# Autodesk Inventor assembly: ChassisComplete_NERDS
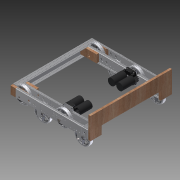
[picture p0: Inventor's stored thumbnail of the model, 180x180]
Saved by Autodesk Inventor 2014 (Build 180170000, 170)
## iProperties
Created: 2016-01-19
Part Number: ChassisComplete_NERDS
Document SubType Name: Assembly
Designer: choices
Author: choices
## Documents named in this file (15)
- C:\Users\choices.CTE\Documents\Nerds_1726\Models\2015-2016\Assemblies\Robot\Chassis.iam
- C:\Users\choices.CTE\Documents\Nerds_1726\Models\2015-2016\AndyMark\6 HiGrip with hub and double pulley.iam
- C:\Users\choices.CTE\Documents\Nerds_1726\Models\2015-2016\AndyMark\FR8ZZ Hex Bearing.ipt
- C:\Users\choices.CTE\Documents\Nerds_1726\Models\2015-2016\AndyMark\am-2598_107 2016 KOP Toughbox Mini.iam
- C:\Users\choices.CTE\Documents\Nerds_1726\Models\2015-2016\AndyMark\6 HiGrip with bearings, pulleys and spacers.iam
- C:\Users\choices.CTE\Documents\Nerds_1726\Models\2015-2016\Parts\Robot\Chassis\FrameInnerRight.ipt
- C:\Users\choices.CTE\Documents\Nerds_1726\Models\2015-2016\AndyMark\375-16 x 4.25 Hex Bolt_HFBOLT 0.375-16x2.5x1-C.ipt
- C:\Users\choices.CTE\Documents\Nerds_1726\Models\2015-2016\Parts\Robot\Chassis\FrameOuterRight.ipt
- C:\Users\choices.CTE\Documents\Nerds_1726\Models\2015-2016\Parts\Robot\Chassis\FrameOuterLeft.ipt
- C:\Users\choices.CTE\Documents\Nerds_1726\Models\2015-2016\Parts\Robot\Chassis\FrameInnerLeft.ipt
- C:\Users\choices.CTE\Documents\Nerds_1726\Models\2015-2016\Parts\Robot\Chassis\DriveFrameEndCaps.ipt
- C:\Users\choices.CTE\Documents\Nerds_1726\Models\2015-2016\Parts\Robot\Chassis\DriveMotor.ipt
- C:\Users\choices.CTE\Documents\Nerds_1726\Models\2015-2016\Parts\Robot\Chassis\BumperMount.ipt
- C:\Users\choices.CTE\Documents\Nerds_1726\Models\2015-2016\Parts\Robot\Chassis\FrameEndSpacer.ipt
- C:\Users\choices.CTE\Documents\Nerds_1726\Models\2015-2016\AndyMark\Chass_EndSheet.ipt
## Components (30 placed, 14 different names)
1. 6 HiGrip with hub and double pulley:1 [sub-assembly] — Mate:7, Mate:8, Mate:9
2. am-2598_107 2016 KOP Toughbox Mini:1 [sub-assembly] — Mate:8, Mate:9, Mate:12, Mate:14, Flush:1, Mate:15, Mate:16, Mate:17, Insert:19, Insert:20
3. FR8ZZ Hex Bearing:1 — Mate:7, Mate:12, Mate:14, Flush:1, Mate:18, Mate:19
4. 6 HiGrip with bearings, pulleys and spacers:1 [sub-assembly] — Insert:5, Tangent:1
5. FrameInnerRight:1 — Mate:15, Mate:16, Mate:17, Insert:5, Insert:6, Insert:8, Flush:2, Mate:39, Mate:40, Flush:11
6. 6 HiGrip with bearings, pulleys and spacers:2 [sub-assembly] — Insert:6
7. 6 HiGrip with bearings, pulleys and spacers:4 [sub-assembly] — Insert:8
8. FrameOuterRight:1 — Mate:18, Mate:19, Insert:9, Flush:3, Mate:29, Mate:31, Mate:32, Mate:37, Mate:38, Flush:10
9. 375-16 x 4.25 Hex Bolt_HFBOLT 0.375-16x2.5x1-C:1 — Insert:9, Tangent:1
10. FrameOuterLeft:1 — Insert:12, Insert:13, Insert:15, Flush:3, Mate:27, Mate:28, Mate:33, Mate:43, Mate:44, Flush:13
11. FrameInnerLeft:1 — Mate:26, Insert:10, Insert:11, Insert:14, Insert:16, Flush:2, Mate:41, Mate:42, Flush:12
12. 6 HiGrip with hub and double pulley:2 [sub-assembly] — Mate:20, Mate:21, Mate:22, Mate:23
13. 6 HiGrip with bearings, pulleys and spacers:5 [sub-assembly] — Insert:13, Tangent:2
14. 6 HiGrip with bearings, pulleys and spacers:6 [sub-assembly] — Insert:15
15. 6 HiGrip with bearings, pulleys and spacers:7 [sub-assembly] — Insert:16
16. am-2598_107 2016 KOP Toughbox Mini:2 [sub-assembly] — Mate:20, Mate:21, Mate:22, Mate:24, Mate:25, Mate:26, Insert:10, Insert:11, Insert:17, Insert:18
17. FR8ZZ Hex Bearing:2 — Mate:23, Mate:24, Mate:25, Insert:12
18. 375-16 x 4.25 Hex Bolt_HFBOLT 0.375-16x2.5x1-C:2 — Insert:14, Tangent:2
19. DriveFrameEndCaps:1 — Mate:29, Mate:31, Mate:32, Mate:35, Flush:6, Flush:15
20. DriveFrameEndCaps:2 — Mate:27, Mate:28, Mate:33, Mate:34, Flush:4, Flush:5
21. DriveMotor:1 — Insert:17
22. DriveMotor:2 — Insert:20
23. DriveMotor:3 — Insert:18
24. DriveMotor:4 — Insert:19
25. BumperMount:1 — Mate:34, Flush:4, Flush:5, Mate:35, Flush:6, Flush:15
26. FrameEndSpacer:1 — Mate:37, Mate:38, Flush:10, Mate:45, Mate:46, Flush:16
27. FrameEndSpacer:2 — Mate:39, Mate:40, Flush:11
28. FrameEndSpacer:3 — Mate:43, Mate:44, Flush:13
29. FrameEndSpacer:4 — Mate:41, Mate:42, Flush:12
30. Chass_EndSheet:1 — Mate:45, Mate:46, Flush:16
## Relationships (64: Mate 35, Insert 15, Flush 12, Tangent 2)
- Mate:7: 6 HiGrip with hub and double pulley:1 ↔ FR8ZZ Hex Bearing:1
- Mate:8: 6 HiGrip with hub and double pulley:1 ↔ am-2598_107 2016 KOP Toughbox Mini:1
- Mate:9: 6 HiGrip with hub and double pulley:1 ↔ am-2598_107 2016 KOP Toughbox Mini:1
- Mate:12: am-2598_107 2016 KOP Toughbox Mini:1 ↔ FR8ZZ Hex Bearing:1
- Mate:14: am-2598_107 2016 KOP Toughbox Mini:1 ↔ FR8ZZ Hex Bearing:1
- Flush:1: am-2598_107 2016 KOP Toughbox Mini:1 ↔ FR8ZZ Hex Bearing:1
- Mate:15: am-2598_107 2016 KOP Toughbox Mini:1 ↔ FrameInnerRight:1
- Mate:16: am-2598_107 2016 KOP Toughbox Mini:1 ↔ FrameInnerRight:1
- Mate:17: am-2598_107 2016 KOP Toughbox Mini:1 ↔ FrameInnerRight:1
- Insert:5: 6 HiGrip with bearings, pulleys and spacers:1 ↔ FrameInnerRight:1
- Insert:6: FrameInnerRight:1 ↔ 6 HiGrip with bearings, pulleys and spacers:2
- Insert:8: FrameInnerRight:1 ↔ 6 HiGrip with bearings, pulleys and spacers:4
- Mate:18: FR8ZZ Hex Bearing:1 ↔ FrameOuterRight:1
- Mate:19: FR8ZZ Hex Bearing:1 ↔ FrameOuterRight:1
- Insert:9: FrameOuterRight:1 ↔ 375-16 x 4.25 Hex Bolt_HFBOLT 0.375-16x2.5x1-C:1
- Tangent:1: 6 HiGrip with bearings, pulleys and spacers:1 ↔ 375-16 x 4.25 Hex Bolt_HFBOLT 0.375-16x2.5x1-C:1
- Mate:20: 6 HiGrip with hub and double pulley:2 ↔ am-2598_107 2016 KOP Toughbox Mini:2
- Mate:21: 6 HiGrip with hub and double pulley:2 ↔ am-2598_107 2016 KOP Toughbox Mini:2
- Mate:22: 6 HiGrip with hub and double pulley:2 ↔ am-2598_107 2016 KOP Toughbox Mini:2
- Mate:23: 6 HiGrip with hub and double pulley:2 ↔ FR8ZZ Hex Bearing:2
- Mate:24: am-2598_107 2016 KOP Toughbox Mini:2 ↔ FR8ZZ Hex Bearing:2
- Mate:25: am-2598_107 2016 KOP Toughbox Mini:2 ↔ FR8ZZ Hex Bearing:2
- Mate:26: FrameInnerLeft:1 ↔ am-2598_107 2016 KOP Toughbox Mini:2
- Insert:10: FrameInnerLeft:1 ↔ am-2598_107 2016 KOP Toughbox Mini:2
- Insert:11: FrameInnerLeft:1 ↔ am-2598_107 2016 KOP Toughbox Mini:2
- Insert:12: FrameOuterLeft:1 ↔ FR8ZZ Hex Bearing:2
- Insert:13: FrameOuterLeft:1 ↔ 6 HiGrip with bearings, pulleys and spacers:5
- Insert:14: FrameInnerLeft:1 ↔ 375-16 x 4.25 Hex Bolt_HFBOLT 0.375-16x2.5x1-C:2
- Tangent:2: 6 HiGrip with bearings, pulleys and spacers:5 ↔ 375-16 x 4.25 Hex Bolt_HFBOLT 0.375-16x2.5x1-C:2
- Insert:15: FrameOuterLeft:1 ↔ 6 HiGrip with bearings, pulleys and spacers:6
- Insert:16: FrameInnerLeft:1 ↔ 6 HiGrip with bearings, pulleys and spacers:7
- Flush:2: FrameInnerRight:1 ↔ FrameInnerLeft:1
- Flush:3: FrameOuterRight:1 ↔ FrameOuterLeft:1
- Mate:27: FrameOuterLeft:1 ↔ DriveFrameEndCaps:2
- Mate:28: FrameOuterLeft:1 ↔ DriveFrameEndCaps:2
- Mate:29: FrameOuterRight:1 ↔ DriveFrameEndCaps:1
- Insert:17: am-2598_107 2016 KOP Toughbox Mini:2 ↔ DriveMotor:1
- Insert:18: am-2598_107 2016 KOP Toughbox Mini:2 ↔ DriveMotor:3
- Insert:19: am-2598_107 2016 KOP Toughbox Mini:1 ↔ DriveMotor:4
- Insert:20: am-2598_107 2016 KOP Toughbox Mini:1 ↔ DriveMotor:2
- Mate:31: FrameOuterRight:1 ↔ DriveFrameEndCaps:1
- Mate:32: FrameOuterRight:1 ↔ DriveFrameEndCaps:1
- Mate:33: FrameOuterLeft:1 ↔ DriveFrameEndCaps:2
- Mate:34: DriveFrameEndCaps:2 ↔ BumperMount:1
- Flush:4: DriveFrameEndCaps:2 ↔ BumperMount:1
- Flush:5: DriveFrameEndCaps:2 ↔ BumperMount:1
- Mate:35: DriveFrameEndCaps:1 ↔ BumperMount:1
- Flush:6: DriveFrameEndCaps:1 ↔ BumperMount:1
- Mate:37: FrameOuterRight:1 ↔ FrameEndSpacer:1
- Mate:38: FrameOuterRight:1 ↔ FrameEndSpacer:1
- Flush:10 (-50.8 mm): FrameOuterRight:1 ↔ FrameEndSpacer:1
- Mate:39: FrameInnerRight:1 ↔ FrameEndSpacer:2
- Mate:40: FrameInnerRight:1 ↔ FrameEndSpacer:2
- Flush:11 (50.8 mm): FrameInnerRight:1 ↔ FrameEndSpacer:2
- Mate:41: FrameInnerLeft:1 ↔ FrameEndSpacer:4
- Mate:42: FrameInnerLeft:1 ↔ FrameEndSpacer:4
- Flush:12 (-50.8 mm): FrameInnerLeft:1 ↔ FrameEndSpacer:4
- Mate:43: FrameOuterLeft:1 ↔ FrameEndSpacer:3
- Mate:44: FrameOuterLeft:1 ↔ FrameEndSpacer:3
- Flush:13 (-50.8 mm): FrameOuterLeft:1 ↔ FrameEndSpacer:3
- Mate:45: FrameEndSpacer:1 ↔ Chass_EndSheet:1
- Mate:46: FrameEndSpacer:1 ↔ Chass_EndSheet:1
- Flush:15: DriveFrameEndCaps:1 ↔ BumperMount:1
- Flush:16: FrameEndSpacer:1 ↔ Chass_EndSheet:1
